# Autodesk Inventor assembly: камера крепить
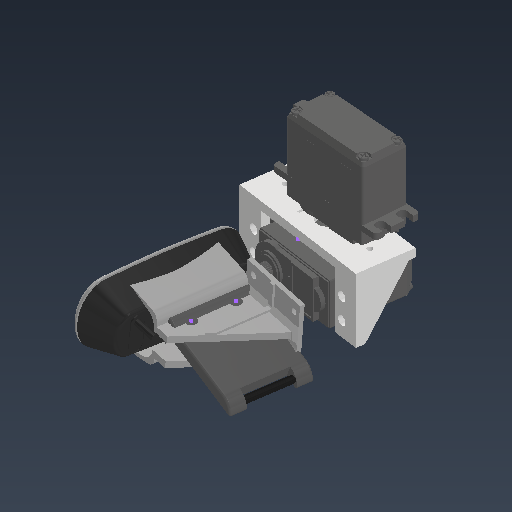
[picture p0: Inventor's stored thumbnail of the model, 512x512]
Saved by Autodesk Inventor 2026 (Build 300175000, 175)
## iProperties
Created: 2026-01-25
Part Number: камера крепить
Document SubType Name: Assembly
Designer: GameHD
Author: GameHD
## Documents named in this file (5)
- C:\Users\GameHD\Desktop\Phantom 16950\камера крепить.iam
- C:\Users\GameHD\Desktop\Phantom 16950\хрень под камеру от глеба (2).ipt
- C:\Users\GameHD\Desktop\Phantom 16950\черт под серву камеру глеба 2 .ipt
- C:\Users\GameHD\Desktop\Phantom 16950\серва мотор.ipt
- C:\Users\GameHD\Desktop\Phantom 16950\genelMontaj\genelMontaj\genelMontaj.iam
## Components (5 placed, 4 different names)
1. хрень под камеру от глеба (2):1 — Совмещение:5, Совмещение:6, Совмещение:7
2. черт под серву камеру глеба 2 :1 — Совмещение:1, Совмещение:2, Совмещение:3, Совмещение:4
3. серва мотор:1 — Совмещение:1, Совмещение:2
4. серва мотор:2 — Совмещение:3, Совмещение:4, Совмещение:5, Совмещение:6
5. genelMontaj:1 [sub-assembly] — Совмещение:7
## Relationships (7: Mate 7)
- Совмещение:1 [Mate]: черт под серву камеру глеба 2 :1 ↔ серва мотор:1
- Совмещение:2 [Mate]: черт под серву камеру глеба 2 :1 ↔ серва мотор:1
- Совмещение:3 [Mate]: черт под серву камеру глеба 2 :1 ↔ серва мотор:2
- Совмещение:4 [Mate]: черт под серву камеру глеба 2 :1 ↔ серва мотор:2
- Совмещение:5 [Mate]: хрень под камеру от глеба (2):1 ↔ серва мотор:2
- Совмещение:6 [Mate]: хрень под камеру от глеба (2):1 ↔ серва мотор:2
- Совмещение:7 [Mate] (5 mm): хрень под камеру от глеба (2):1 ↔ genelMontaj:1
